# Autodesk Inventor assembly: gear-stack-big
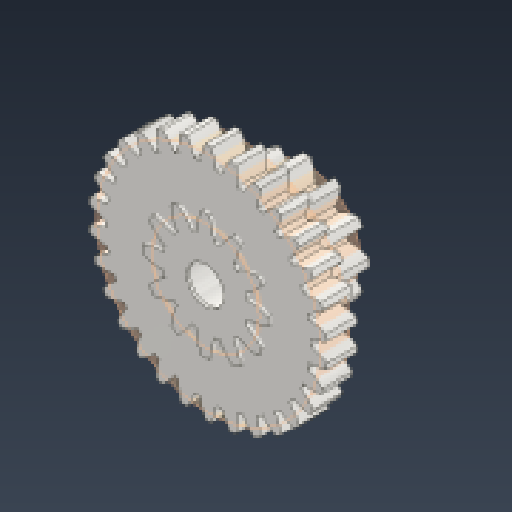
[picture p0: Inventor's stored thumbnail of the model, 512x512]
Saved by Autodesk Inventor 2023 (Build 270158000, 158)
## iProperties
Created: 2025-04-27
Part Number: gear-stack-big
Document SubType Name: Assembly
Designer: szymo
Mass: 4 g
Surface Area: 9.80478 cm^2
Volume: 0.58347 cm^3
Author: szymo
## Documents named in this file (3)
- D:\tech\robotyka\robots\evangelion-turbo\inventor-project\gear-stack-big.iam
- D:\tech\robotyka\robots\evangelion-turbo\inventor-project\gear-stack-big\Design Accelerator\Spur Gears1.iam
- D:\tech\robotyka\robots\evangelion-turbo\inventor-project\gear-stack-big\Design Accelerator\Spur Gears2.iam
## Components (2 placed, 1 different names)
1. Spur Gears:1 [sub-assembly] — Mate:1, Flush:1, Mate:2, Mate:3, Mate:4, Flush:2, Angle:1, Angle:2, Angle:3
2. Spur Gears:2 [sub-assembly] — Mate:1, Flush:1, Mate:2
## Relationships (9: Mate 4, Angle 3, Flush 2)
- Mate:1: Spur Gears:1 ↔ Spur Gears:2
- Flush:1 (0.2 mm): Spur Gears:1 ↔ Spur Gears:2
- Mate:2: Spur Gears:1 ↔ Spur Gears:2
- Mate:3: Spur Gears:1
- Mate:4: Spur Gears:1
- Flush:2: Spur Gears:1
- Angle:1 (180 deg): Spur Gears:1
- Angle:2 (180 deg): Spur Gears:1
- Angle:3 (0 deg): Spur Gears:1
